# Autodesk Inventor assembly: batterycart assemble
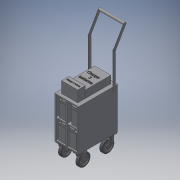
[picture p0: Inventor's stored thumbnail of the model, 180x180]
Saved by Autodesk Inventor 2019 (Build 230136000, 136)
## iProperties
Created: 2018-12-09
Part Number: batterycart assemble
Document SubType Name: Assembly
Designer: Tiberus
Author: Tiberus
## Documents named in this file (7)
- C:\Users\Tiberus\Documents\Inventor\Robotics\batterycart assemble.iam
- C:\Users\Tiberus\Documents\Inventor\Robotics\battery charger 2019.ipt
- C:\Users\Tiberus\Documents\Inventor\Robotics\batterycart skeleton.ipt
- C:\Users\Tiberus\Downloads\AIS2019\2_05456_444.iam
- C:\Users\Tiberus\Documents\Inventor\Robotics\1 battery charger 2019.ipt
- C:\Users\Tiberus\Documents\Inventor\Robotics\cart handle.ipt
- C:\Users\Tiberus\Downloads\BatteryModel.ipt
## Components (16 placed, 6 different names)
1. battery charger 2019:1 — Mate:17, Flush:9, Flush:10
2. batterycart skeleton:1 — Mate:17, Mate:18, Mate:19, Mate:20, Mate:21, Flush:1, Flush:2, Flush:3, Flush:4, Flush:5, Flush:6, Flush:7, Flush:8, Flush:9, Flush:10, Mate:22, Flush:11, Flush:12, Mate:23, Mate:24, Mate:25, Mate:26, Mate:27, Mate:28, Mate:29, Mate:30, Mate:31, Mate:32, Mate:33, Mate:34, Mate:35, Mate:36, Mate:37, Mate:38, Mate:39
3. 2_05456_444:1 [sub-assembly] — Mate:21, Flush:7, Flush:8
4. 2_05456_444:2 [sub-assembly] — Mate:20, Flush:5, Flush:6
5. 2_05456_444:3 [sub-assembly] — Mate:19, Flush:1, Flush:2
6. 2_05456_444:4 [sub-assembly] — Mate:18, Flush:3, Flush:4
7. 1 battery charger 2019:1 — Mate:22, Flush:11, Flush:12
8. cart handle:1 — Mate:23
9. BatteryModel:1 — Mate:26, Mate:27
10. BatteryModel:2 — Mate:28, Mate:29
11. BatteryModel:3 — Mate:30, Mate:31
12. BatteryModel:4 — Mate:36, Mate:37
13. BatteryModel:5 — Mate:38, Mate:39
14. BatteryModel:6 — Mate:34, Mate:35
15. BatteryModel:7 — Mate:24, Mate:25
16. BatteryModel:8 — Mate:32, Mate:33
## Relationships (35: Mate 23, Flush 12)
- Mate:17: battery charger 2019:1 ↔ batterycart skeleton:1
- Mate:18: batterycart skeleton:1 ↔ 2_05456_444:4
- Mate:19: batterycart skeleton:1 ↔ 2_05456_444:3
- Mate:20: batterycart skeleton:1 ↔ 2_05456_444:2
- Mate:21: batterycart skeleton:1 ↔ 2_05456_444:1
- Flush:1: batterycart skeleton:1 ↔ 2_05456_444:3
- Flush:2: batterycart skeleton:1 ↔ 2_05456_444:3
- Flush:3: batterycart skeleton:1 ↔ 2_05456_444:4
- Flush:4: batterycart skeleton:1 ↔ 2_05456_444:4
- Flush:5: batterycart skeleton:1 ↔ 2_05456_444:2
- Flush:6: batterycart skeleton:1 ↔ 2_05456_444:2
- Flush:7: batterycart skeleton:1 ↔ 2_05456_444:1
- Flush:8: batterycart skeleton:1 ↔ 2_05456_444:1
- Flush:9 (38.1 mm): battery charger 2019:1 ↔ batterycart skeleton:1
- Flush:10 (31.115 mm): battery charger 2019:1 ↔ batterycart skeleton:1
- Mate:22: batterycart skeleton:1 ↔ 1 battery charger 2019:1
- Flush:11 (31.115 mm): batterycart skeleton:1 ↔ 1 battery charger 2019:1
- Flush:12 (38.1 mm): batterycart skeleton:1 ↔ 1 battery charger 2019:1
- Mate:23: batterycart skeleton:1 ↔ cart handle:1
- Mate:24: batterycart skeleton:1 ↔ BatteryModel:7
- Mate:25: batterycart skeleton:1 ↔ BatteryModel:7
- Mate:26: batterycart skeleton:1 ↔ BatteryModel:1
- Mate:27: batterycart skeleton:1 ↔ BatteryModel:1
- Mate:28: batterycart skeleton:1 ↔ BatteryModel:2
- Mate:29: batterycart skeleton:1 ↔ BatteryModel:2
- Mate:30: batterycart skeleton:1 ↔ BatteryModel:3
- Mate:31: batterycart skeleton:1 ↔ BatteryModel:3
- Mate:32: batterycart skeleton:1 ↔ BatteryModel:8
- Mate:33: batterycart skeleton:1 ↔ BatteryModel:8
- Mate:34: batterycart skeleton:1 ↔ BatteryModel:6
- Mate:35: batterycart skeleton:1 ↔ BatteryModel:6
- Mate:36: batterycart skeleton:1 ↔ BatteryModel:4
- Mate:37: batterycart skeleton:1 ↔ BatteryModel:4
- Mate:38: batterycart skeleton:1 ↔ BatteryModel:5
- Mate:39: batterycart skeleton:1 ↔ BatteryModel:5
